# Autodesk Inventor assembly: Laser Galvo Assembly
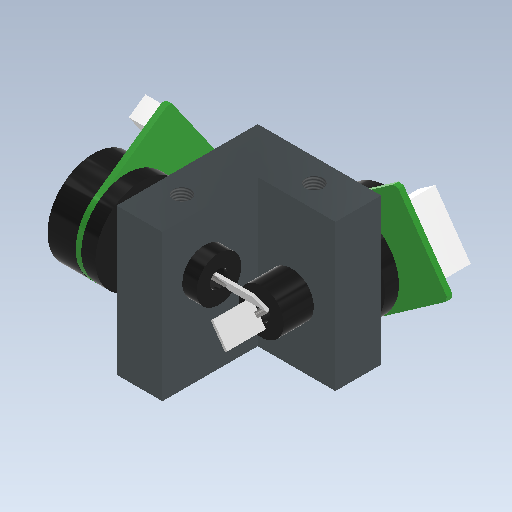
[picture p0: Inventor's stored thumbnail of the model, 512x512]
Saved by Autodesk Inventor 2021 (Build 250183000, 183)
## iProperties
Created: 2021-04-06
Part Number: Laser Galvo Assembly
Document SubType Name: Assembly
Designer: Andrew
Author: Andrew
## Documents named in this file (3)
- D:\Projects\school\Spring 2021\CECS490A\CAD\Laser Galvo Assembly.iam
- D:\Projects\school\Spring 2021\CECS490A\CAD\AT 25-5246.ipt
- D:\Projects\school\Spring 2021\CECS490A\CAD\Laser Galvo Mount.ipt
## Components (3 placed, 2 different names)
1. Laser Galvo Mount:1 — Flush:1, Flush:2, Flush:3, Mate:1, Mate:2, Mate:3, Mate:4, Angle:1, Angle:2
2. AT 25-5246:1 — Mate:2, Mate:4, Angle:2
3. AT 25-5246:2 — Mate:1, Mate:3, Angle:1
## Relationships (9: Mate 4, Flush 3, Angle 2)
- Flush:1: Laser Galvo Mount:1
- Flush:2: Laser Galvo Mount:1
- Flush:3: Laser Galvo Mount:1
- Mate:1: Laser Galvo Mount:1 ↔ AT 25-5246:2
- Mate:2: Laser Galvo Mount:1 ↔ AT 25-5246:1
- Mate:3 (0.5 mm): Laser Galvo Mount:1 ↔ AT 25-5246:2
- Mate:4 (5 mm): Laser Galvo Mount:1 ↔ AT 25-5246:1
- Angle:1 (35 deg): Laser Galvo Mount:1 ↔ AT 25-5246:2
- Angle:2 (-35 deg): Laser Galvo Mount:1 ↔ AT 25-5246:1
